# Autodesk Inventor assembly: FrontGearboxAssembly
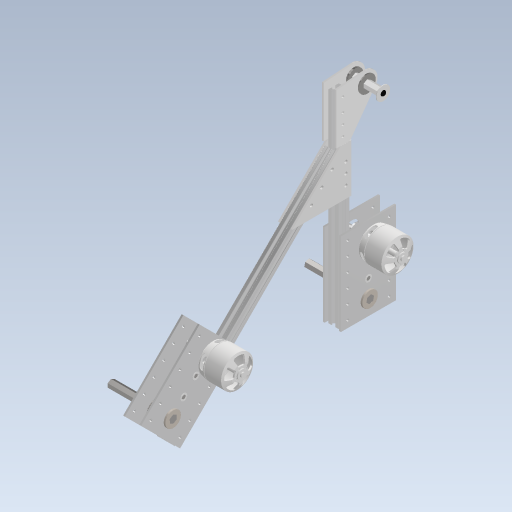
[picture p0: Inventor's stored thumbnail of the model, 512x512]
Saved by Autodesk Inventor 2023 (Build 270158000, 158)
## iProperties
Created: 2023-02-14
Part Number: FrontGearboxAssembly
Document SubType Name: Assembly
Designer: Dave
Author: Dave
## Documents named in this file (7)
- C:\Users\Dave\Documents\GitHub\BehrendURCMechanical\CAD\Chassis\GearBox\Final Gears and Assemblies\FrontGearboxAssembly.iam
- C:\Users\Dave\Documents\GitHub\BehrendURCMechanical\CAD\Chassis\GearBox\Final Gears and Assemblies\Gearbox Assembly.iam
- C:\Users\Dave\Documents\GitHub\BehrendURCMechanical\CAD\Chassis\CH-1-01-FrontKneeJoint.ipt
- C:\Users\Dave\Documents\GitHub\BehrendURCMechanical\CAD\Chassis\HipJoint.iam
- C:\Users\Dave\Documents\GitHub\BehrendURCMechanical\CAD\Chassis\CH-1-01-20x20 Channel.ipt
- C:\Users\Dave\Documents\GitHub\BehrendURCMechanical\CAD\Chassis\CH-1-01-20x20 Channel\CH-1-01-20x20 Channel-372.ipt
- C:\Users\Dave\Documents\GitHub\BehrendURCMechanical\CAD\Chassis\CH-1-01-20x20 Channel\CH-1-01-20x20 Channel-437.ipt
## Components (7 placed, 5 different names)
1. Gearbox Assembly:1 [sub-assembly] — Angle:1, Flush:1, Angle:2, Tangent:1, Flush:13, Mate:15, Flush:18, Flush:19
2. Gearbox Assembly:2 [sub-assembly] — Flush:1, Angle:2, Flush:21
3. CH-1-01-FrontKneeJoint:1 — Flush:11, Flush:12, Mate:19
4. HipJoint:1 [sub-assembly] — Mate:18, Mate:22, Tangent:2
5. CH-1-01-FrontKneeJoint:2 — Flush:11, Flush:12, Mate:18, Flush:14, Flush:20
6. CH-1-01-20x20 Channel-437:1 — Mate:19, Flush:14, Flush:17, Flush:21
7. CH-1-01-20x20 Channel-372:2 — Flush:17, Mate:22, Flush:18, Flush:19, Tangent:2, Flush:20
## Relationships (18: Flush 10, Mate 4, Angle 2, Tangent 2)
- Angle:1 (90 deg): Gearbox Assembly:1
- Flush:1: Gearbox Assembly:1 ↔ Gearbox Assembly:2
- Angle:2 (-45 deg): Gearbox Assembly:1 ↔ Gearbox Assembly:2
- Tangent:1: Gearbox Assembly:1
- Flush:11: CH-1-01-FrontKneeJoint:1 ↔ CH-1-01-FrontKneeJoint:2
- Flush:12: CH-1-01-FrontKneeJoint:1 ↔ CH-1-01-FrontKneeJoint:2
- Flush:13: Gearbox Assembly:1
- Mate:15: Gearbox Assembly:1
- Mate:18: HipJoint:1 ↔ CH-1-01-FrontKneeJoint:2
- Mate:19: CH-1-01-FrontKneeJoint:1 ↔ CH-1-01-20x20 Channel-437:1
- Flush:14: CH-1-01-FrontKneeJoint:2 ↔ CH-1-01-20x20 Channel-437:1
- Flush:17: CH-1-01-20x20 Channel-437:1 ↔ CH-1-01-20x20 Channel-372:2
- Mate:22: HipJoint:1 ↔ CH-1-01-20x20 Channel-372:2
- Flush:18: Gearbox Assembly:1 ↔ CH-1-01-20x20 Channel-372:2
- Flush:19 (2.6924 mm): Gearbox Assembly:1 ↔ CH-1-01-20x20 Channel-372:2
- Tangent:2: HipJoint:1 ↔ CH-1-01-20x20 Channel-372:2
- Flush:20: CH-1-01-FrontKneeJoint:2 ↔ CH-1-01-20x20 Channel-372:2
- Flush:21 (-2.6924 mm): Gearbox Assembly:2 ↔ CH-1-01-20x20 Channel-437:1
